# Autodesk Inventor assembly: Pendulum
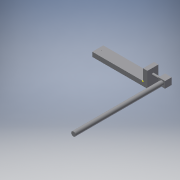
[picture p0: Inventor's stored thumbnail of the model, 180x180]
Saved by Autodesk Inventor 2016 (Build 200138000, 138)
## iProperties
Created: 2015-10-29
Part Number: Pendulum
Document SubType Name: Assembly
Designer: nightstalker
Mass: 455.707 g
Surface Area: 787.22 cm^2
Volume: 455.707 cm^3
Density: 1 g/cm^3
Author: nightstalker
## Documents named in this file (6)
- G:\Miscellaneous\Work\UMD Assignments\ENPM 808M - Exam 1\Assembly\Pendulum.iam
- G:\Miscellaneous\Work\UMD Assignments\ENPM 808M - Exam 1\Parts\A.ipt
- G:\Miscellaneous\Work\UMD Assignments\ENPM 808M - Exam 1\Parts\B.ipt
- G:\Miscellaneous\Work\UMD Assignments\ENPM 808M - Exam 1\Parts\C.ipt
- G:\Miscellaneous\Work\UMD Assignments\ENPM 808M - Exam 1\Parts\D.ipt
- G:\Miscellaneous\Work\UMD Assignments\ENPM 808M - Exam 1\Parts\E.ipt
## Components (5 placed, 5 different names)
1. A:1 — Rigid:1
2. B:1 — Rigid:1, Rotational:1
3. C:1 — Rigid:2, Rigid:3
4. D:1 — Rigid:2
5. E:1 — Rigid:3, Rotational:1
## Relationships (4: WeldJoint 3, RevoluteJoint 1)
- Rigid:1 [WeldJoint]: A:1 ↔ B:1
- Rigid:2 [WeldJoint]: C:1 ↔ D:1
- Rigid:3 [WeldJoint]: C:1 ↔ E:1
- Rotational:1 [RevoluteJoint]: B:1 ↔ E:1
